# Autodesk Inventor assembly: Vertical Support Assembly
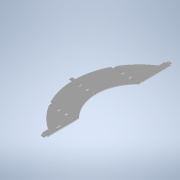
[picture p0: Inventor's stored thumbnail of the model, 180x180]
Saved by Autodesk Inventor 2021 (Build 250183000, 183)
## iProperties
Created: 2020-07-30
Part Number: Vertical Support Assembly
Document SubType Name: Assembly
Designer: Dan Wikman
Author: Dan Wikman
## Documents named in this file (5)
- C:\Users\danny\OneDrive\University Life\2020, Semester 1\METR4900 Honours Thesis\PROTOTYPE V2\Vertical Support Assembly.iam
- C:\Users\danny\OneDrive\University Life\2020, Semester 1\METR4900 Honours Thesis\PROTOTYPE V2\Support A - V2.ipt
- C:\Users\danny\OneDrive\University Life\2020, Semester 1\METR4900 Honours Thesis\PROTOTYPE V2\Support B - V2.ipt
- C:\Users\danny\OneDrive\University Life\2020, Semester 1\METR4900 Honours Thesis\PROTOTYPE V2\Support C - V2.ipt
- C:\Users\danny\OneDrive\University Life\2020, Semester 1\METR4900 Honours Thesis\PROTOTYPE V2\Support D - V2.ipt
## Components (4 placed, 4 different names)
1. Support A - V2:1 — Flush:3, Mate:9, Flush:7
2. Support B - V2:1 — Flush:2, Flush:3, Mate:8, Mate:9, Flush:7, Flush:8
3. Support C - V2:1 — Flush:2, Flush:4, Flush:5, Mate:8, Flush:8, Mate:10
4. Support D - V2:1 — Flush:4, Flush:5, Mate:10
## Relationships (9: Flush 6, Mate 3)
- Flush:2: Support B - V2:1 ↔ Support C - V2:1
- Flush:3: Support A - V2:1 ↔ Support B - V2:1
- Flush:4: Support C - V2:1 ↔ Support D - V2:1
- Flush:5: Support C - V2:1 ↔ Support D - V2:1
- Mate:8: Support B - V2:1 ↔ Support C - V2:1
- Mate:9: Support A - V2:1 ↔ Support B - V2:1
- Flush:7: Support A - V2:1 ↔ Support B - V2:1
- Flush:8: Support B - V2:1 ↔ Support C - V2:1
- Mate:10: Support C - V2:1 ↔ Support D - V2:1
